# Autodesk Inventor assembly: Gear
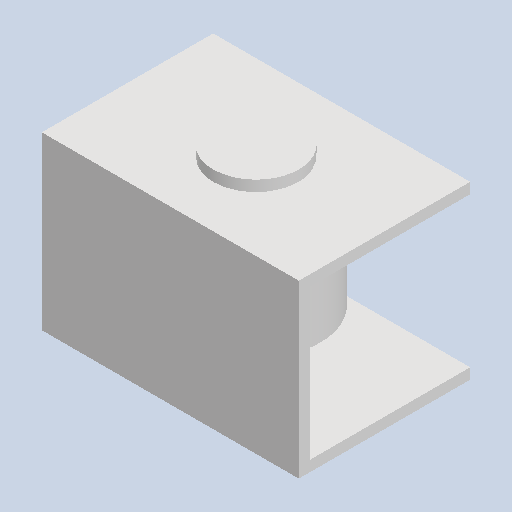
[picture p0: Inventor's stored thumbnail of the model, 512x512]
Saved by Autodesk Inventor 2023 (Build 270158030, 158C)
## iProperties
Created: 2023-02-13
Part Number: Gear
Document SubType Name: Assembly
Designer: jeremyy
Author: jeremyy
## Documents named in this file (3)
- \\andrew.ad.cmu.edu\users\users1\jeremyy\Documents\Inventor\CMU Bridge\New folder\Gear.iam
- \\andrew.ad.cmu.edu\users\users1\jeremyy\Documents\Inventor\CMU Bridge\New folder\Gear Shell.ipt
- \\andrew.ad.cmu.edu\users\users1\jeremyy\Documents\Inventor\CMU Bridge\New folder\Gear Wheel.ipt
## Components (2 placed, 2 different names)
1. Gear Shell:1 — Tangent:1, Mate:1
2. Gear Wheel:1 — Tangent:1, Mate:1
## Relationships (2: Tangent 1, Mate 1)
- Tangent:1: Gear Shell:1 ↔ Gear Wheel:1
- Mate:1: Gear Shell:1 ↔ Gear Wheel:1
